# Autodesk Inventor assembly: Thigh-40x
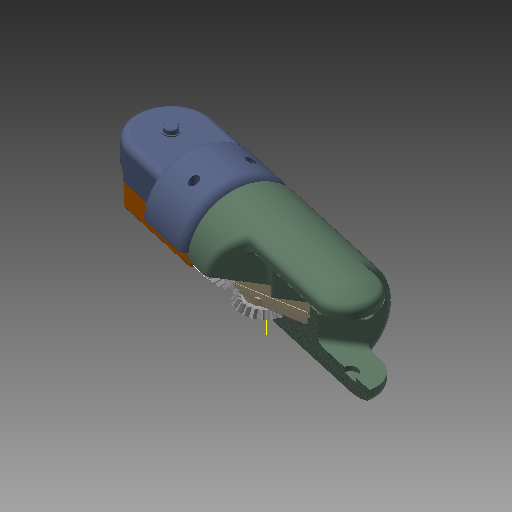
[picture p0: Inventor's stored thumbnail of the model, 512x512]
Saved by Autodesk Inventor 2018 (Build 220112000, 112)
## iProperties
Part Number: Thigh-40x
Material: Generisch
Document SubType Name: Assembly
Designer: Jochen Alt
Mass: 186.402 g
Surface Area: 1060.57 cm^2
Volume: 140.56 cm^3
Density: 1.32614 g/cm^3
Author: Jochen Alt
## Documents named in this file (11)
- D:\Projects\Manfred\design\cad\Inventor\Thigh-40x.iam
- D:\Projects\Manfred\design\cad\Inventor\Herkulex DRS-010x\W 61707-2RS1.ipt
- D:\Projects\Manfred\design\cad\Inventor\Rillenkugellager 11x7x3 inafag smr117.ipt
- D:\Projects\Manfred\design\cad\Inventor\Thigh-40x.ipt
- D:\Projects\Manfred\design\cad\Inventor\Herkulex DRS-040x.ipt
- D:\Projects\Manfred\design\cad\Inventor\Knee-40x.ipt
- D:\Projects\Manfred\design\cad\Inventor\Herkulex DRS-010x\HerkuleX DRS-0101.iam
- D:\Projects\Manfred\design\cad\Inventor\Thigh Bushing 040x.ipt
- D:\Projects\Manfred\design\cad\Inventor\ThighKneeGear.iam
- C:\Users\JochenAlt\Documents\Inventor\Content Center Files\R2018\de-DE\ISO 4762(1)\DIN EN ISO 4762 - M2,5 x 4.ipt
- C:\Users\JochenAlt\Documents\Inventor\Content Center Files\R2018\de-DE\ISO 4762(1)\DIN EN ISO 4762 - M2 x 3.ipt
## Components (18 placed, 10 different names)
1. W 61707-2RS1:1 — Passend:44, Passend:54, Passend:73, Passend:74
2. Rillenkugellager 11x7x3 inafag smr117:2 — Passend:78, Passend:79
3. Thigh-40x:1 — Passend:44, Passend:54, Winkel:2, Fluchtend:1, Passend:64, Winkel:3, Passend:75, Passend:77, Winkel:5, Passend:83, Einfügen:1, Einfügen:2, Einfügen:3, Einfügen:4
4. Herkulex DRS-040x:1 — Winkel:2, Fluchtend:1, Passend:64
5. Knee-40x:1 — Passend:75, Winkel:4, Passend:82, Passend:84, Einfügen:5, Einfügen:6, Einfügen:7, Einfügen:8, Einfügen:9, Einfügen:10
6. HerkuleX DRS-0101:1 [sub-assembly] — Winkel:4, Passend:80, Passend:81
7. Thigh Bushing 040x:1 — Passend:73, Passend:74, Passend:76, Passend:84
8. ThighKneeGear:1 [sub-assembly] — Passend:76, Passend:77, Winkel:5, Passend:78, Passend:79, Passend:80, Passend:81, Passend:82, Passend:83
9. DIN EN ISO 4762 M2,5 x 4:1 — Einfügen:1
10. DIN EN ISO 4762 M2,5 x 4:2 — Einfügen:2
11. DIN EN ISO 4762 M2,5 x 4:3 — Einfügen:3
12. DIN EN ISO 4762 M2,5 x 4:4 — Einfügen:4
13. DIN EN ISO 4762 M2 x 3:1 — Einfügen:5
14. DIN EN ISO 4762 M2 x 3:2 — Einfügen:6
15. DIN EN ISO 4762 M2 x 3:3 — Einfügen:7
16. DIN EN ISO 4762 M2 x 3:4 — Einfügen:8
17. DIN EN ISO 4762 M2 x 3:5 — Einfügen:9
18. DIN EN ISO 4762 M2 x 3:6 — Einfügen:10
## Relationships (30: Mate 15, Insert 10, Angle 4, Flush 1)
- Passend:44 [Mate]: W 61707-2RS1:1 ↔ Thigh-40x:1
- Passend:54 [Mate]: W 61707-2RS1:1 ↔ Thigh-40x:1
- Winkel:2 [Angle] (180 deg): Thigh-40x:1 ↔ Herkulex DRS-040x:1
- Fluchtend:1 [Flush] (0.2 mm): Thigh-40x:1 ↔ Herkulex DRS-040x:1
- Passend:64 [Mate]: Thigh-40x:1 ↔ Herkulex DRS-040x:1
- Winkel:3 [Angle] (0 deg): Thigh-40x:1
- Passend:73 [Mate]: W 61707-2RS1:1 ↔ Thigh Bushing 040x:1
- Passend:74 [Mate] (0.1 mm): W 61707-2RS1:1 ↔ Thigh Bushing 040x:1
- Passend:75 [Mate]: Thigh-40x:1 ↔ Knee-40x:1
- Winkel:4 [Angle] (180 deg): Knee-40x:1 ↔ HerkuleX DRS-0101:1
- Passend:76 [Mate]: Thigh Bushing 040x:1 ↔ ThighKneeGear:1
- Passend:77 [Mate] (0.1 mm): Thigh-40x:1 ↔ ThighKneeGear:1
- Winkel:5 [Angle] (180 deg): Thigh-40x:1 ↔ ThighKneeGear:1
- Passend:78 [Mate]: Rillenkugellager 11x7x3 inafag smr117:2 ↔ ThighKneeGear:1
- Passend:79 [Mate]: Rillenkugellager 11x7x3 inafag smr117:2 ↔ ThighKneeGear:1
- Passend:80 [Mate]: HerkuleX DRS-0101:1 ↔ ThighKneeGear:1
- Passend:81 [Mate] (0.1 mm): HerkuleX DRS-0101:1 ↔ ThighKneeGear:1
- Passend:82 [Mate]: Knee-40x:1 ↔ ThighKneeGear:1
- Passend:83 [Mate] (0.1 mm): Thigh-40x:1 ↔ ThighKneeGear:1
- Passend:84 [Mate]: Knee-40x:1 ↔ Thigh Bushing 040x:1
- Einfügen:1 [Insert]: Thigh-40x:1 ↔ DIN EN ISO 4762 M2,5 x 4:1
- Einfügen:2 [Insert]: Thigh-40x:1 ↔ DIN EN ISO 4762 M2,5 x 4:2
- Einfügen:3 [Insert]: Thigh-40x:1 ↔ DIN EN ISO 4762 M2,5 x 4:3
- Einfügen:4 [Insert]: Thigh-40x:1 ↔ DIN EN ISO 4762 M2,5 x 4:4
- Einfügen:5 [Insert]: Knee-40x:1 ↔ DIN EN ISO 4762 M2 x 3:1
- Einfügen:6 [Insert]: Knee-40x:1 ↔ DIN EN ISO 4762 M2 x 3:2
- Einfügen:7 [Insert]: Knee-40x:1 ↔ DIN EN ISO 4762 M2 x 3:3
- Einfügen:8 [Insert]: Knee-40x:1 ↔ DIN EN ISO 4762 M2 x 3:4
- Einfügen:9 [Insert]: Knee-40x:1 ↔ DIN EN ISO 4762 M2 x 3:5
- Einfügen:10 [Insert]: Knee-40x:1 ↔ DIN EN ISO 4762 M2 x 3:6
